# Autodesk Inventor assembly: Assembly_Guinardia_V1
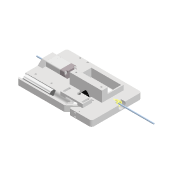
[picture p0: Inventor's stored thumbnail of the model, 180x180]
Saved by Autodesk Inventor 2022 (Build 260153000, 153)
## iProperties
Created: 2022-04-18
Part Number: Assembly_Guinardia_V1
Document SubType Name: Assembly
Designer: Prakash Lab
Author: Prakash Lab
## Documents named in this file (10)
- C:\Users\UC2\Documents\GitHub\Guinardia\INVENTOR\Assembly_Guinardia_V1.iam
- C:\Users\UC2\Documents\GitHub\Guinardia\INVENTOR\00_NEMA8.ipt
- C:\Users\UC2\Documents\GitHub\Guinardia\INVENTOR\00_CCTV_lens_M12_25mm_5mp.ipt
- C:\Users\UC2\Documents\GitHub\Guinardia\INVENTOR\00_coverslip_24x50mm.ipt
- C:\Users\UC2\Documents\GitHub\Guinardia\INVENTOR\00_PipetteTip200ul-1.ipt
- C:\Users\UC2\Documents\GitHub\Guinardia\INVENTOR\00_FEP_tube_2.2x0.5mm.ipt
- C:\Users\UC2\Documents\GitHub\Guinardia\INVENTOR\00_Bluraymirror_6.4x6.4x2mm.ipt
- C:\Users\UC2\Documents\GitHub\Guinardia\INVENTOR\00_Laserpointer.ipt
- C:\Users\UC2\Documents\GitHub\Guinardia\INVENTOR\10_LED_cylnderlensmount.ipt
- C:\Users\UC2\Documents\GitHub\Guinardia\INVENTOR\10_Wellplate_base_v1.ipt
## Components (11 placed, 9 different names)
1. 10_Wellplate_base_v1:1 — Mate:1, Mate:2, Mate:3, Mate:4, Mate:5, Flush:1, Mate:10, Flush:2, Mate:11, Mate:12, Insert:1, Flush:10, Flush:11, Einfügen:2
2. 00_CCTV_lens_M12_25mm_5mp:1 — Mate:6, Flush:1
3. 00_coverslip_24x50mm:1 — Mate:1, Mate:2, Mate:3, Mate:7, Mate:13
4. 00_PipetteTip200ul-1:2 — Mate:9, Flush:2
5. 00_FEP_tube_2.2x0.5mm:1 — Mate:4, Mate:5, Mate:8, Mate:9, Mate:7
6. 00_PipetteTip200ul-1:3 — Mate:8, Mate:6, Mate:10
7. 00_coverslip_24x50mm:2 — Mate:11, Mate:12, Mate:13
8. 00_Bluraymirror_6.4x6.4x2mm:1
9. 00_Laserpointer:1 — Insert:1
10. 10_LED_cylnderlensmount:1 — Flush:10, Flush:11
11. 00_NEMA8:1 — Einfügen:2
## Relationships (19: Mate 13, Flush 4, Insert 2)
- Mate:1: 10_Wellplate_base_v1:1 ↔ 00_coverslip_24x50mm:1
- Mate:2: 10_Wellplate_base_v1:1 ↔ 00_coverslip_24x50mm:1
- Mate:3: 10_Wellplate_base_v1:1 ↔ 00_coverslip_24x50mm:1
- Mate:4 (-6 mm): 10_Wellplate_base_v1:1 ↔ 00_FEP_tube_2.2x0.5mm:1
- Mate:5: 10_Wellplate_base_v1:1 ↔ 00_FEP_tube_2.2x0.5mm:1
- Mate:8: 00_FEP_tube_2.2x0.5mm:1 ↔ 00_PipetteTip200ul-1:3
- Mate:9: 00_PipetteTip200ul-1:2 ↔ 00_FEP_tube_2.2x0.5mm:1
- Mate:6: 00_CCTV_lens_M12_25mm_5mp:1 ↔ 00_PipetteTip200ul-1:3
- Flush:1: 10_Wellplate_base_v1:1 ↔ 00_CCTV_lens_M12_25mm_5mp:1
- Mate:7 (3 mm): 00_coverslip_24x50mm:1 ↔ 00_FEP_tube_2.2x0.5mm:1
- Mate:10 (4 mm): 10_Wellplate_base_v1:1 ↔ 00_PipetteTip200ul-1:3
- Flush:2 (5 mm): 10_Wellplate_base_v1:1 ↔ 00_PipetteTip200ul-1:2
- Mate:11: 10_Wellplate_base_v1:1 ↔ 00_coverslip_24x50mm:2
- Mate:12: 10_Wellplate_base_v1:1 ↔ 00_coverslip_24x50mm:2
- Mate:13: 00_coverslip_24x50mm:1 ↔ 00_coverslip_24x50mm:2
- Insert:1: 10_Wellplate_base_v1:1 ↔ 00_Laserpointer:1
- Flush:10: 10_Wellplate_base_v1:1 ↔ 10_LED_cylnderlensmount:1
- Flush:11: 10_Wellplate_base_v1:1 ↔ 10_LED_cylnderlensmount:1
- Einfügen:2 [Insert]: 10_Wellplate_base_v1:1 ↔ 00_NEMA8:1
